# Autodesk Inventor assembly: tip_3_n_base
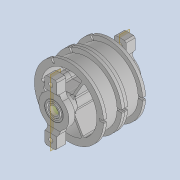
[picture p0: Inventor's stored thumbnail of the model, 180x180]
Saved by Autodesk Inventor 2020 (Build 240168000, 168)
## iProperties
Created: 2021-10-07
Part Number: tip_3_n_base
Document SubType Name: Assembly
Designer: Shuang Peng
Author: Shuang Peng
## Documents named in this file (4)
- D:\projects-3\torque fb tip\hardware\tip_3\tip_3_n_base.iam
- D:\projects-3\torque fb tip\hardware\tip_3\roller_4.ipt
- D:\projects-3\torque fb tip\hardware\tip_3\bearing_hh_1.ipt
- D:\projects-3\torque fb tip\hardware\tip_3\bearing_3_6_2.ipt
## Components (6 placed, 3 different names)
1. roller_4:1 — Insert:1, Insert:5
2. roller_4:2 — Insert:1, Insert:4
3. bearing_hh_1:1 — Insert:3, Flush:1
4. bearing_hh_1:2 — Insert:2, Flush:1
5. bearing_3_6_2:1 — Insert:2, Insert:5
6. bearing_3_6_2:2 — Insert:3, Insert:4
## Relationships (6: Insert 5, Flush 1)
- Insert:1: roller_4:1 ↔ roller_4:2
- Insert:2: bearing_hh_1:2 ↔ bearing_3_6_2:1
- Insert:3: bearing_hh_1:1 ↔ bearing_3_6_2:2
- Insert:4: roller_4:2 ↔ bearing_3_6_2:2
- Insert:5: roller_4:1 ↔ bearing_3_6_2:1
- Flush:1: bearing_hh_1:1 ↔ bearing_hh_1:2
